# Autodesk Inventor assembly: Telaio - Trasporto
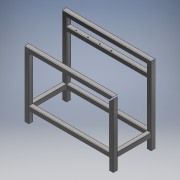
[picture p0: Inventor's stored thumbnail of the model, 180x180]
Saved by Autodesk Inventor 2018 (Build 220112000, 112)
## iProperties
Created: 2020-05-30
Part Number: Telaio - Trasporto
Material: Generico
Document SubType Name: Weldment
Designer: Francesco
Weld Material: Welded Aluminum-6061
Author: Francesco
## Documents named in this file (7)
- C:\Users\Francesco\no-brim\Meccanica\Progetto Inventor no-brim\Assiemi\Telaio - Trasporto.iam
- C:\Users\Francesco\no-brim\Meccanica\Progetto Inventor no-brim\Parti\Piantone tubolare l magg.ipt
- C:\Users\Francesco\no-brim\Meccanica\Progetto Inventor no-brim\Parti\Tubolari horizontal superiore.ipt
- C:\Users\Francesco\no-brim\Meccanica\Progetto Inventor no-brim\Parti\Tubolari horizontal 45 rulliera.ipt
- C:\Users\Francesco\no-brim\Meccanica\Progetto Inventor no-brim\Parti\Piantone tubolare l min.ipt
- C:\Users\Francesco\no-brim\Meccanica\Progetto Inventor no-brim\Parti\Tubolare horizontal corto.ipt
- C:\Users\Francesco\no-brim\Meccanica\Progetto Inventor no-brim\Parti\Tubolari horizontal.ipt
## Components (11 placed, 5 different names)
1. Piantone tubolare l magg:1 — Coincidente:1, Allineato:1, Allineato:3, Allineato:7, Allineato:8, Coincidente:9, Allineato:12, Allineato:16
2. Piantone tubolare l magg:2 — Coincidente:2, Allineato:2, Allineato:3, Coincidente:3, Allineato:4, Coincidente:4, Allineato:5, Allineato:6, Coincidente:11, Allineato:14, Coincidente:12
3. Tubolari horizontal:1 — Coincidente:1, Allineato:1, Coincidente:2, Allineato:2, Coincidente:5
4. Tubolari horizontal 45:1 — Coincidente:3, Allineato:4, Coincidente:4, Coincidente:5
5. Piantone tubolare l min:1 — Allineato:7, Allineato:8, Allineato:9, Coincidente:10, Allineato:18
6. Piantone tubolare l min:2 — Allineato:5, Allineato:6, Allineato:9, Coincidente:6, Coincidente:7, Allineato:10, Coincidente:8, Allineato:11
7. Tubolari horizontal 45:2 — Coincidente:6, Coincidente:7, Allineato:10
8. Tubolare horizontal corto:1 — Coincidente:11, Allineato:14, Allineato:15
9. Tubolare horizontal corto:2 — Coincidente:9, Allineato:12, Allineato:13, Coincidente:10, Allineato:17
10. Tubolari horizontal:2 — Coincidente:12, Allineato:16, Allineato:17
11. Tubolari horizontal:3 — Coincidente:8, Allineato:11, Allineato:13, Allineato:15, Allineato:18
## Relationships (30: Flush 18, Mate 12)
- Coincidente:1 [Mate]: Piantone tubolare l magg:1 ↔ Tubolari horizontal:1
- Allineato:1 [Flush]: Piantone tubolare l magg:1 ↔ Tubolari horizontal:1
- Coincidente:2 [Mate]: Piantone tubolare l magg:2 ↔ Tubolari horizontal:1
- Allineato:2 [Flush]: Piantone tubolare l magg:2 ↔ Tubolari horizontal:1
- Allineato:3 [Flush]: Piantone tubolare l magg:1 ↔ Piantone tubolare l magg:2
- Coincidente:3 [Mate]: Piantone tubolare l magg:2 ↔ Tubolari horizontal 45:1
- Allineato:4 [Flush]: Piantone tubolare l magg:2 ↔ Tubolari horizontal 45:1
- Coincidente:4 [Mate]: Piantone tubolare l magg:2 ↔ Tubolari horizontal 45:1
- Coincidente:5 [Mate] (70 mm): Tubolari horizontal:1 ↔ Tubolari horizontal 45:1
- Allineato:5 [Flush]: Piantone tubolare l magg:2 ↔ Piantone tubolare l min:2
- Allineato:6 [Flush]: Piantone tubolare l magg:2 ↔ Piantone tubolare l min:2
- Allineato:7 [Flush]: Piantone tubolare l magg:1 ↔ Piantone tubolare l min:1
- Allineato:8 [Flush]: Piantone tubolare l magg:1 ↔ Piantone tubolare l min:1
- Allineato:9 [Flush]: Piantone tubolare l min:1 ↔ Piantone tubolare l min:2
- Coincidente:6 [Mate]: Piantone tubolare l min:2 ↔ Tubolari horizontal 45:2
- Coincidente:7 [Mate]: Piantone tubolare l min:2 ↔ Tubolari horizontal 45:2
- Allineato:10 [Flush]: Piantone tubolare l min:2 ↔ Tubolari horizontal 45:2
- Coincidente:8 [Mate]: Piantone tubolare l min:2 ↔ Tubolari horizontal:3
- Allineato:11 [Flush]: Piantone tubolare l min:2 ↔ Tubolari horizontal:3
- Coincidente:9 [Mate]: Piantone tubolare l magg:1 ↔ Tubolare horizontal corto:2
- Allineato:12 [Flush]: Piantone tubolare l magg:1 ↔ Tubolare horizontal corto:2
- Allineato:13 [Flush]: Tubolare horizontal corto:2 ↔ Tubolari horizontal:3
- Coincidente:10 [Mate]: Piantone tubolare l min:1 ↔ Tubolare horizontal corto:2
- Coincidente:11 [Mate]: Piantone tubolare l magg:2 ↔ Tubolare horizontal corto:1
- Allineato:14 [Flush]: Piantone tubolare l magg:2 ↔ Tubolare horizontal corto:1
- Allineato:15 [Flush]: Tubolare horizontal corto:1 ↔ Tubolari horizontal:3
- Coincidente:12 [Mate]: Piantone tubolare l magg:2 ↔ Tubolari horizontal:2
- Allineato:16 [Flush]: Piantone tubolare l magg:1 ↔ Tubolari horizontal:2
- Allineato:17 [Flush]: Tubolare horizontal corto:2 ↔ Tubolari horizontal:2
- Allineato:18 [Flush] (-100 mm): Piantone tubolare l min:1 ↔ Tubolari horizontal:3
